# Autodesk Inventor assembly: MG-Dribblingmotor v2
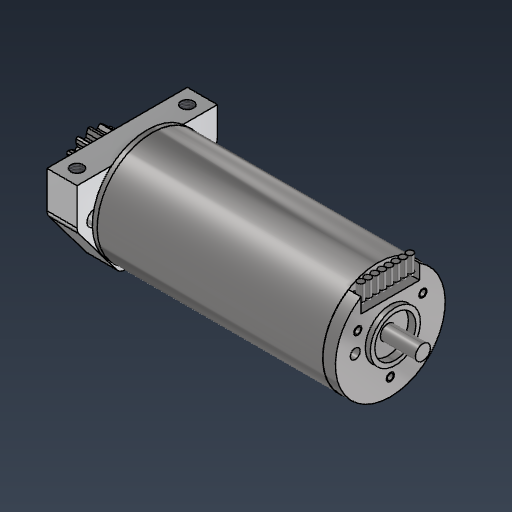
[picture p0: Inventor's stored thumbnail of the model, 512x512]
Saved by Autodesk Inventor 2023.1 (Build 271208000, 208)
## iProperties
Part Number: MG-Dribblingmotor v2
Material: Generisch
Document SubType Name: Assembly
Designer: rYan
Mass: 141.194 g
Surface Area: 72.0618 cm^2
Volume: 20.8403 cm^3
Author: rYan
## Documents named in this file (5)
- D:\TIGERsGIT\Hardware\mechanik\2024\Inventor\Robot\Dribbler\MG-Dribblingmotor v2.iam
- D:\TIGERsGIT\Hardware\mechanik\2024\Inventor\Robot\Dribbler\Motorhalter.ipt
- D:\TIGERsGIT\Hardware\mechanik\2024\Inventor\Purchased Parts\MaxonECmax22-25W.ipt
- D:\TIGERsGIT\Hardware\mechanik\2024\Inventor\Inhaltscenter\de-DE\ISO 4762(2)\ISO 4762 - M2 x 6ISO.ipt
- D:\TIGERsGIT\Hardware\mechanik\2024\Inventor\Purchased Parts\Zahnrad z14 Modul 0.7 Motor.ipt
## Components (6 placed, 4 different names)
1. Motorhalter:1 — Passend:1, Passend:2, Fluchtend:1, Einfügen:2, Passend:6, Einfügen:3, Einfügen:4, Einfügen:5
2. MaxonECmax22-25W:1 — Einfügen:2, Passend:6, Einfügen:6
3. ISO 4762 M2 x 6:1 — Einfügen:4
4. ISO 4762 M2 x 6:2 — Einfügen:5
5. ISO 4762 M2 x 6:3 — Einfügen:3
6. Zahnrad z14 Modul 0.7 Motor:1 — Einfügen:6
## Relationships (9: Insert 5, Mate 3, Flush 1)
- Passend:1 [Mate]: Motorhalter:1
- Passend:2 [Mate]: Motorhalter:1
- Fluchtend:1 [Flush]: Motorhalter:1
- Einfügen:2 [Insert]: Motorhalter:1 ↔ MaxonECmax22-25W:1
- Passend:6 [Mate]: Motorhalter:1 ↔ MaxonECmax22-25W:1
- Einfügen:3 [Insert]: Motorhalter:1 ↔ ISO 4762 M2 x 6:3
- Einfügen:4 [Insert]: Motorhalter:1 ↔ ISO 4762 M2 x 6:1
- Einfügen:5 [Insert]: Motorhalter:1 ↔ ISO 4762 M2 x 6:2
- Einfügen:6 [Insert] (-1.6 mm): MaxonECmax22-25W:1 ↔ Zahnrad z14 Modul 0.7 Motor:1
